# Autodesk Inventor assembly: tensioner
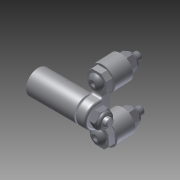
[picture p0: Inventor's stored thumbnail of the model, 180x180]
Saved by Autodesk Inventor 2014 SP1 (Build 180222100, 222)
## iProperties
Created: 2013-08-29
Part Number: tensioner
Document SubType Name: Assembly
Designer: Ryan
Sending System: SolidWorks 2013
Last Author: Ryan
Author: Ryan
## Documents named in this file (7)
- C:\Users\Ryan\Desktop\sw\toss up 4th robot\drive\pillow block tensioner.iam
- C:\Users\Ryan\Desktop\sw\lib\Aperture VEX CAD Library\Spacers\SPACER-0500-0500.ipt
- C:\Users\Ryan\Desktop\sw\lib\Aperture VEX CAD Library\Hardware\8-32\8-32 Nylock.ipt
- C:\Users\Ryan\Desktop\sw\lib\Aperture VEX CAD Library\Bearing Blocks\Pillow Block.ipt
- C:\Users\Ryan\Desktop\sw\lib\Aperture VEX CAD Library\Hardware\8-32\8-32_1.500.ipt
- C:\Users\Ryan\Desktop\sw\lib\Aperture VEX CAD Library\Spacers\SPACER-0500-0375.ipt
- C:\Users\Ryan\Desktop\sw\lib\Aperture VEX CAD Library\Hardware\8-32\8-32_.875.ipt
## Components (11 placed, 7 different names)
1. 8-32_1-000:1
2. spacer-0500-0500:1 — Mate:5, Mate:6
3. 8-32 nylock:1 — Mate:7, Mate:11
4. SPACER-0500-0500:2 — Mate:5, Mate:6, Mate:7, Mate:12
5. Pillow Block:1 — Mate:11, Mate:12, Mate:13, Mate:14, Mate:15, Mate:16, Mate:20, Mate:21, Mate:22
6. SPACER-0500-0375:1 — Mate:13, Mate:14
7. SPACER-0500-0375:2 — Mate:15, Mate:16, Mate:19, Mate:24
8. 8-32_.875:2 — Mate:21, Mate:22, Mate:25
9. 8-32_.875:1 — Mate:19, Mate:20, Mate:23
10. 8-32 nylock:2 — Flush:1, Mate:25
11. 8-32 nylock:3 — Flush:1, Mate:23, Mate:24
## Relationships (20: Mate 19, Flush 1)
- Mate:5: spacer-0500-0500:1 ↔ SPACER-0500-0500:2
- Mate:6: spacer-0500-0500:1 ↔ SPACER-0500-0500:2
- Mate:7: 8-32 nylock:1 ↔ SPACER-0500-0500:2
- [Mate]: 8-32_1-000:1 ↔ spacer-0500-0500:1
- [Mate]: 8-32_1-000:1 ↔ spacer-0500-0500:1
- [Mate]: 8-32_1-000:1 ↔ Pillow Block:1
- Mate:11: 8-32 nylock:1 ↔ Pillow Block:1
- Mate:12: SPACER-0500-0500:2 ↔ Pillow Block:1
- Mate:13: Pillow Block:1 ↔ SPACER-0500-0375:1
- Mate:14: Pillow Block:1 ↔ SPACER-0500-0375:1
- Mate:15: Pillow Block:1 ↔ SPACER-0500-0375:2
- Mate:16: Pillow Block:1 ↔ SPACER-0500-0375:2
- Mate:19: SPACER-0500-0375:2 ↔ 8-32_.875:1
- Mate:20: Pillow Block:1 ↔ 8-32_.875:1
- Mate:21: Pillow Block:1 ↔ 8-32_.875:2
- Mate:22: Pillow Block:1 ↔ 8-32_.875:2
- Flush:1: 8-32 nylock:2 ↔ 8-32 nylock:3
- Mate:23: 8-32_.875:1 ↔ 8-32 nylock:3
- Mate:24 (1.1684 mm): SPACER-0500-0375:2 ↔ 8-32 nylock:3
- Mate:25: 8-32_.875:2 ↔ 8-32 nylock:2
